# Autodesk Inventor assembly: toggle switch cover
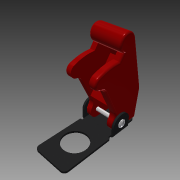
[picture p0: Inventor's stored thumbnail of the model, 180x180]
Saved by Autodesk Inventor 2012 (Build 160160000, 160)
## iProperties
Created: 2014-01-27
Part Number: toggle switch cover
Document SubType Name: Assembly
Designer: Michał
Author: Michał
## Documents named in this file (4)
- G:\Moje Dokumenty\Inventor\toggle switch cover\toggle switch cover.iam
- G:\Moje Dokumenty\Inventor\toggle switch cover\01.ipt
- G:\Moje Dokumenty\Inventor\toggle switch cover\02.ipt
- G:\Moje Dokumenty\Inventor\toggle switch cover\03.ipt
## Components (3 placed, 3 different names)
1. 01:1 — Insert:1, Insert:2
2. 02:1 — Insert:2
3. 03:1 — Insert:1
## Relationships (2: Insert 2)
- Insert:1 (0.25 mm): 01:1 ↔ 03:1
- Insert:2: 01:1 ↔ 02:1
